# Autodesk Inventor assembly: Leg_joint_yaw_frame_WearingImage
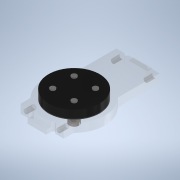
[picture p0: Inventor's stored thumbnail of the model, 180x180]
Saved by Autodesk Inventor 2020.4 (Build 244396000, 396)
## iProperties
Created: 2022-03-16
Part Number: Leg_joint_yaw_frame_WearingImage
Document SubType Name: Assembly
Designer: Masato Kubotera
Author: Masato Kubotera
## Documents named in this file (4)
- C:\Users\Masato\Documents\Inventor\CIT Brains_Inventor\SUSTAINA-OP\SandBlastingJig\Leg_joint_yaw_frame_WearingImage.iam
- C:\Users\Masato\Documents\Inventor\CIT Brains_Inventor\SUSTAINA-OP\LowerBody\Leg_joit\Leg_joint_yaw_frame.ipt
- C:\Users\Masato\Documents\Inventor\CIT Brains_Inventor\SUSTAINA-OP\SandBlastingJig\Leg_joint_yaw_frame_SandBlastingJig.ipt
- C:\Users\Masato\Documents\Inventor\CIT Brains_Inventor\SUSTAINA-OP\ReadyMade\Screw\M3-10.ipt
## Components (6 placed, 3 different names)
1. Leg_joint_yaw_frame:1 — 挿入:1, 挿入:2, 挿入:3, 挿入:4, 挿入:5, 挿入:6, 挿入:7
2. Leg_joint_yaw_frame_SandBlastingJig:1 — 挿入:1, 挿入:2, 挿入:3
3. M3-10:1 — 挿入:4
4. M3-10:2 — 挿入:5
5. M3-10:3 — 挿入:6
6. M3-10:4 — 挿入:7
## Relationships (7: Insert 7)
- 挿入:1 [Insert]: Leg_joint_yaw_frame:1 ↔ Leg_joint_yaw_frame_SandBlastingJig:1
- 挿入:2 [Insert]: Leg_joint_yaw_frame:1 ↔ Leg_joint_yaw_frame_SandBlastingJig:1
- 挿入:3 [Insert]: Leg_joint_yaw_frame:1 ↔ Leg_joint_yaw_frame_SandBlastingJig:1
- 挿入:4 [Insert]: Leg_joint_yaw_frame:1 ↔ M3-10:1
- 挿入:5 [Insert]: Leg_joint_yaw_frame:1 ↔ M3-10:2
- 挿入:6 [Insert]: Leg_joint_yaw_frame:1 ↔ M3-10:3
- 挿入:7 [Insert]: Leg_joint_yaw_frame:1 ↔ M3-10:4
